# Autodesk Inventor assembly: SERVO
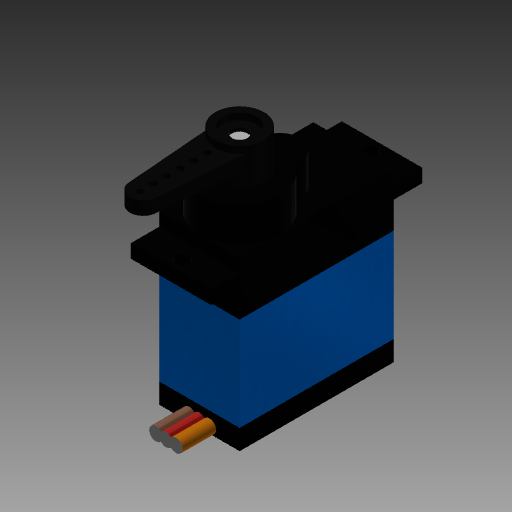
[picture p0: Inventor's stored thumbnail of the model, 512x512]
Saved by Autodesk Inventor 2017 (Build 210142000, 142)
## iProperties
Created: 2017-09-24
Part Number: SERVO
Document SubType Name: Assembly
Designer: Alexander Miller
Author: Alexander Miller
## Documents named in this file (3)
- D:\Daten\Documents\Git\HeRo-Mini\Hardware\SERVO.iam
- D:\Daten\Documents\Git\HeRo-Mini\Hardware\TP-MG92B.ipt
- D:\Daten\Documents\Git\HeRo-Mini\Hardware\TP-MG92B_HAT.ipt
## Components (2 placed, 2 different names)
1. TP-MG92B:1 — Rotational:1
2. TP-MG92B_HAT:1 — Rotational:1
## Relationships (1: RevoluteJoint 1)
- Rotational:1 [RevoluteJoint]: TP-MG92B:1 ↔ TP-MG92B_HAT:1
